# Autodesk Inventor assembly: Idler Front-Unit [A]
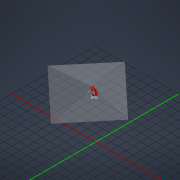
[picture p0: Inventor's stored thumbnail of the model, 180x180]
Saved by Autodesk Inventor 2022.2 (Build 262287010, 287A)
## iProperties
Created: 2022-03-14
Part Number: Idler Front-Unit [A]
Document SubType Name: Assembly
Designer: sleib
Author: sleib
## Documents named in this file (11)
- C:\Users\sleib\Projekte\Voron-2\CAD\Inventor\Idler Front-Unit [A].iam
- C:\Users\sleib\Projekte\Voron-2\CAD\Inventor\Idler Front Bottom [A].ipt
- C:\Users\sleib\Projekte\Voron-2\CAD\Inventor\Idler Front Top [A].ipt
- C:\Users\sleib\Projekte\Voron-2\CAD\Inventor\Idler Front Tensioner-Unit [A].iam
- C:\Users\sleib\Projekte\Voron-2\CAD\Inventor\M3x40 SHCS.ipt
- C:\Users\sleib\Projekte\Voron-2\CAD\Inventor\M5 Spacer (1mm).ipt
- C:\Users\sleib\Projekte\Voron-2\CAD\Inventor\Bearing F695-ZZ.ipt
- C:\Users\sleib\Projekte\Voron-2\CAD\Inventor\Z Belt-Clamp Upper.ipt
- C:\Users\sleib\Projekte\Voron-2\CAD\Inventor\M5x16 BHCS.ipt
- C:\Users\sleib\Projekte\Voron-2\CAD\Inventor\M3 Washer.ipt
- C:\Users\sleib\Projekte\Voron-2\CAD\Inventor\Camera-Unit.iam
## Components (13 placed, 10 different names)
1. Idler Front Bottom [A]:1 — Fluchtend:2, Passend:26, Passend:1, Passend:2, Passend:3, Fluchtend:4, Passend:4, Winkel:1, Passend:6, Passend:14, Passend:24
2. Idler Front Top [A]:1 — Passend:2, Passend:3, Fluchtend:4, Passend:18, Passend:19, Passend:20
3. M3x40 SHCS:1 — Passend:4, Passend:5, Passend:23, Passend:25
4. Idler Front Tensioner-Unit [A]:1 [sub-assembly] — Passend:5, Winkel:1, Passend:6, Passend:7, Passend:8, Passend:9, Passend:10
5. M5 Spacer (1mm):1 — Passend:7, Passend:11
6. M5 Spacer (1mm):2 — Passend:10, Passend:13, Passend:14
7. Bearing F695-ZZ:1 — Passend:9, Passend:11, Passend:12
8. Bearing F695-ZZ:2 — Passend:8, Passend:12, Passend:13
9. Z Belt-Clamp Upper:1 — Passend:16, Passend:17, Passend:20, Passend:21, Passend:22, Passend:27, Fluchtend:5, Fluchtend:6
10. M5x16 BHCS:1 — Passend:16, Passend:19, Passend:22
11. M5x16 BHCS:2 — Passend:17, Passend:18, Passend:21
12. M3 Washer:1 — Passend:23, Passend:24, Passend:25
13. Camera-Unit:1 [sub-assembly] — Passend:27, Fluchtend:5, Fluchtend:6
## Relationships (31: Mate 26, Flush 4, Angle 1)
- Fluchtend:2 [Flush]: Idler Front Bottom [A]:1
- Passend:26 [Mate]: Idler Front Bottom [A]:1
- Passend:1 [Mate]: Idler Front Bottom [A]:1
- Passend:2 [Mate]: Idler Front Bottom [A]:1 ↔ Idler Front Top [A]:1
- Passend:3 [Mate]: Idler Front Bottom [A]:1 ↔ Idler Front Top [A]:1
- Fluchtend:4 [Flush]: Idler Front Bottom [A]:1 ↔ Idler Front Top [A]:1
- Passend:4 [Mate]: Idler Front Bottom [A]:1 ↔ M3x40 SHCS:1
- Passend:5 [Mate]: M3x40 SHCS:1 ↔ Idler Front Tensioner-Unit [A]:1
- Winkel:1 [Angle] (0 deg): Idler Front Bottom [A]:1 ↔ Idler Front Tensioner-Unit [A]:1
- Passend:6 [Mate] (5 mm): Idler Front Bottom [A]:1 ↔ Idler Front Tensioner-Unit [A]:1
- Passend:7 [Mate]: Idler Front Tensioner-Unit [A]:1 ↔ M5 Spacer (1mm):1
- Passend:8 [Mate]: Idler Front Tensioner-Unit [A]:1 ↔ Bearing F695-ZZ:2
- Passend:9 [Mate]: Idler Front Tensioner-Unit [A]:1 ↔ Bearing F695-ZZ:1
- Passend:10 [Mate]: Idler Front Tensioner-Unit [A]:1 ↔ M5 Spacer (1mm):2
- Passend:11 [Mate]: M5 Spacer (1mm):1 ↔ Bearing F695-ZZ:1
- Passend:12 [Mate]: Bearing F695-ZZ:1 ↔ Bearing F695-ZZ:2
- Passend:13 [Mate]: M5 Spacer (1mm):2 ↔ Bearing F695-ZZ:2
- Passend:14 [Mate]: Idler Front Bottom [A]:1 ↔ M5 Spacer (1mm):2
- Passend:16 [Mate]: Z Belt-Clamp Upper:1 ↔ M5x16 BHCS:1
- Passend:17 [Mate]: Z Belt-Clamp Upper:1 ↔ M5x16 BHCS:2
- Passend:18 [Mate]: Idler Front Top [A]:1 ↔ M5x16 BHCS:2
- Passend:19 [Mate]: Idler Front Top [A]:1 ↔ M5x16 BHCS:1
- Passend:20 [Mate]: Idler Front Top [A]:1 ↔ Z Belt-Clamp Upper:1
- Passend:21 [Mate]: Z Belt-Clamp Upper:1 ↔ M5x16 BHCS:2
- Passend:22 [Mate]: Z Belt-Clamp Upper:1 ↔ M5x16 BHCS:1
- Passend:23 [Mate]: M3x40 SHCS:1 ↔ M3 Washer:1
- Passend:24 [Mate]: Idler Front Bottom [A]:1 ↔ M3 Washer:1
- Passend:25 [Mate]: M3x40 SHCS:1 ↔ M3 Washer:1
- Passend:27 [Mate]: Z Belt-Clamp Upper:1 ↔ Camera-Unit:1
- Fluchtend:5 [Flush] (1 mm): Z Belt-Clamp Upper:1 ↔ Camera-Unit:1
- Fluchtend:6 [Flush]: Z Belt-Clamp Upper:1 ↔ Camera-Unit:1
